# Autodesk Inventor assembly: moulding_assembly
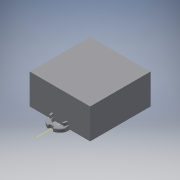
[picture p0: Inventor's stored thumbnail of the model, 180x180]
Saved by Autodesk Inventor 2017 (Build 210142000, 142)
## iProperties
Created: 2018-06-01
Part Number: moulding_assembly
Document SubType Name: Assembly
Designer: Nic
Author: Nic
## Documents named in this file (3)
- C:\Users\Nic\Documents\Antenna\moulding_assembly.iam
- C:\Users\Nic\Documents\Antenna\mould_casing.ipt
- C:\Users\Nic\Documents\Antenna\middle_segment.ipt
## Components (2 placed, 2 different names)
1. middle_segment:1 — Insert:1, Angle:1
2. mould_casing:1 — Insert:1, Angle:1, Mate:1, Mate:2
## Relationships (5: Mate 3, Insert 1, Angle 1)
- Insert:1: middle_segment:1 ↔ mould_casing:1
- Angle:1 (0 deg): middle_segment:1 ↔ mould_casing:1
- Mate:1: mould_casing:1
- Mate:2: mould_casing:1
- Mate:4
